# Autodesk Inventor assembly: Electronics Cover Assembly
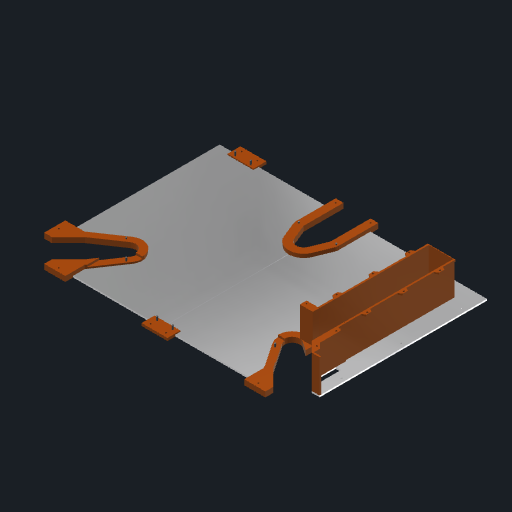
[picture p0: Inventor's stored thumbnail of the model, 512x512]
Saved by Autodesk Inventor 2023.3 (Build 273359000, 359)
## iProperties
Created: 2023-02-24
Part Number: Electronics Cover Assembly
Document SubType Name: Assembly
Designer: remop
Author: remop
## Documents named in this file (10)
- C:\Users\remop\OneDrive\Documents\Inventor\3D Printers\LuEVO\Mk5_FullKinematic\Frame and Panels\Electronics Cover\Electronics Cover Assembly.iam
- C:\Users\remop\OneDrive\Documents\Inventor\3D Printers\LuEVO\Mk5_FullKinematic\Frame and Panels\Electronics Cover\Front Left Cover Bracket.ipt
- C:\Users\remop\OneDrive\Documents\Inventor\3D Printers\LuEVO\Mk5_FullKinematic\Frame and Panels\Electronics Cover\Front Right Cover Bracket.ipt
- C:\Users\remop\OneDrive\Documents\Inventor\3D Printers\LuEVO\Mk5_FullKinematic\Frame and Panels\Electronics Cover\Rear Cover Bracket.ipt
- C:\Users\remop\OneDrive\Documents\Inventor\3D Printers\LuEVO\Mk5_FullKinematic\Frame and Panels\Electronics Cover\Beam Cover Bracket.ipt
- C:\Users\remop\OneDrive\Documents\Inventor\3D Printers\LuEVO\Mk5_FullKinematic\Frame and Panels\Electronics Cover\Electronics Cover Panel.ipt
- C:\Users\remop\OneDrive\Documents\Inventor\3D Printers\LuEVO\Mk5_FullKinematic\Frame and Panels\Electronics Cover\Drag Chain Cover Panel.ipt
- C:\Users\remop\OneDrive\Documents\Inventor\Content Center Files\R2023\en-US\AS 1420\AS 1420 - 1973 - M3 x 12.ipt
- C:\Users\remop\OneDrive\Documents\Inventor\3D Printers\LuEVO\Mk5_FullKinematic\Frame and Panels\Electronics Cover\Drag Chain Cover.ipt
- C:\Users\remop\OneDrive\Documents\Inventor\3D Printers\LuEVO\Mk5_FullKinematic\Frame and Panels\Electronics Cover\Drag Chain Edge Panel.ipt
## Components (22 placed, 9 different names)
1. Front Left Cover Bracket:1 — Flush:1, Flush:2, Mate:1, Flush:3, Flush:4, Flush:5, Flush:8
2. Front Right Cover Bracket:1 — Flush:1, Flush:2, Mate:1, Flush:11
3. Rear Cover Bracket:1 — Flush:3, Mate:2, Flush:6, Flush:7
4. Beam Cover Bracket:1 — Flush:4, Flush:5, Mate:2, Flush:12
5. Beam Cover Bracket:2 — Flush:6, Flush:7, Flush:8, Flush:9, Flush:10
6. Beam Cover Bracket:3 — Flush:9, Flush:10, Flush:11
7. Electronics Cover Panel:1 — Flush:12, Insert:1, Insert:2, Insert:3, Insert:4, Insert:5, Insert:6, Insert:7, Insert:8, Insert:9, Insert:10, Insert:11, Insert:12
8. Drag Chain Cover Panel:1 — Flush:13, Flush:14, Mate:3, Flush:15
9. AS 1420 - Metric M3 x 12:1 — Insert:1
10. AS 1420 - Metric M3 x 12:2 — Insert:2
11. AS 1420 - Metric M3 x 12:3 — Insert:3
12. AS 1420 - Metric M3 x 12:4 — Insert:4
13. AS 1420 - Metric M3 x 12:5 — Insert:5
14. AS 1420 - Metric M3 x 12:6 — Insert:6
15. AS 1420 - Metric M3 x 12:7 — Insert:7
16. AS 1420 - Metric M3 x 12:8 — Insert:8
17. AS 1420 - Metric M3 x 12:9 — Insert:9
18. AS 1420 - Metric M3 x 12:10 — Insert:10
19. AS 1420 - Metric M3 x 12:11 — Insert:11
20. AS 1420 - Metric M3 x 12:12 — Insert:12
21. Drag Chain Cover:1 — Flush:13, Flush:14, Mate:3
22. Drag Chain Edge Panel:1 — Flush:15
## Relationships (30: Flush 15, Insert 12, Mate 3)
- Flush:1: Front Left Cover Bracket:1 ↔ Front Right Cover Bracket:1
- Flush:2: Front Left Cover Bracket:1 ↔ Front Right Cover Bracket:1
- Mate:1 (344.5 mm): Front Left Cover Bracket:1 ↔ Front Right Cover Bracket:1
- Flush:3: Front Left Cover Bracket:1 ↔ Rear Cover Bracket:1
- Flush:4: Front Left Cover Bracket:1 ↔ Beam Cover Bracket:1
- Flush:5: Front Left Cover Bracket:1 ↔ Beam Cover Bracket:1
- Mate:2 (1.063 mm): Rear Cover Bracket:1 ↔ Beam Cover Bracket:1
- Flush:6: Rear Cover Bracket:1 ↔ Beam Cover Bracket:2
- Flush:7: Rear Cover Bracket:1 ↔ Beam Cover Bracket:2
- Flush:8 (5 mm): Front Left Cover Bracket:1 ↔ Beam Cover Bracket:2
- Flush:9: Beam Cover Bracket:2 ↔ Beam Cover Bracket:3
- Flush:10: Beam Cover Bracket:2 ↔ Beam Cover Bracket:3
- Flush:11 (40 mm): Front Right Cover Bracket:1 ↔ Beam Cover Bracket:3
- Flush:12: Beam Cover Bracket:1 ↔ Electronics Cover Panel:1
- Insert:1: Electronics Cover Panel:1 ↔ AS 1420 - Metric M3 x 12:1
- Insert:2: Electronics Cover Panel:1 ↔ AS 1420 - Metric M3 x 12:2
- Insert:3: Electronics Cover Panel:1 ↔ AS 1420 - Metric M3 x 12:3
- Insert:4: Electronics Cover Panel:1 ↔ AS 1420 - Metric M3 x 12:4
- Insert:5: Electronics Cover Panel:1 ↔ AS 1420 - Metric M3 x 12:5
- Insert:6: Electronics Cover Panel:1 ↔ AS 1420 - Metric M3 x 12:6
- Insert:7: Electronics Cover Panel:1 ↔ AS 1420 - Metric M3 x 12:7
- Insert:8: Electronics Cover Panel:1 ↔ AS 1420 - Metric M3 x 12:8
- Insert:9: Electronics Cover Panel:1 ↔ AS 1420 - Metric M3 x 12:9
- Insert:10: Electronics Cover Panel:1 ↔ AS 1420 - Metric M3 x 12:10
- Insert:11: Electronics Cover Panel:1 ↔ AS 1420 - Metric M3 x 12:11
- Insert:12: Electronics Cover Panel:1 ↔ AS 1420 - Metric M3 x 12:12
- Flush:13: Drag Chain Cover Panel:1 ↔ Drag Chain Cover:1
- Flush:14: Drag Chain Cover Panel:1 ↔ Drag Chain Cover:1
- Mate:3: Drag Chain Cover Panel:1 ↔ Drag Chain Cover:1
- Flush:15: Drag Chain Cover Panel:1 ↔ Drag Chain Edge Panel:1
